# Autodesk Inventor assembly: main room with double door
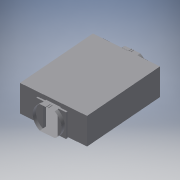
[picture p0: Inventor's stored thumbnail of the model, 180x180]
Saved by Autodesk Inventor 2017 (Build 210142000, 142)
## iProperties
Created: 2018-03-03
Part Number: main room with double door
Document SubType Name: Assembly
Designer: Braxton
Author: Braxton
## Documents named in this file (3)
- E:\School\Game develpment\geoscape\done (one wall)\rooms  (one wall)\assembly\main room with double door.iam
- E:\School\Game develpment\geoscape\done (one wall)\rooms  (one wall)\starting room (one wall).ipt
- E:\School\Game develpment\geoscape\done (one wall)\doors\double door.ipt
## Components (3 placed, 2 different names)
1. starting room (one wall):1 — Mate:1, Mate:2, Mate:3, Mate:4, Mate:5, Mate:6
2. double door:1 — Mate:2, Mate:3, Mate:6
3. double door:2 — Mate:1, Mate:4, Mate:5
## Relationships (6: Mate 6)
- Mate:1: starting room (one wall):1 ↔ double door:2
- Mate:2: starting room (one wall):1 ↔ double door:1
- Mate:3: starting room (one wall):1 ↔ double door:1
- Mate:4: starting room (one wall):1 ↔ double door:2
- Mate:5: starting room (one wall):1 ↔ double door:2
- Mate:6: starting room (one wall):1 ↔ double door:1
